# Autodesk Inventor assembly: PS MW RSP-2000-48
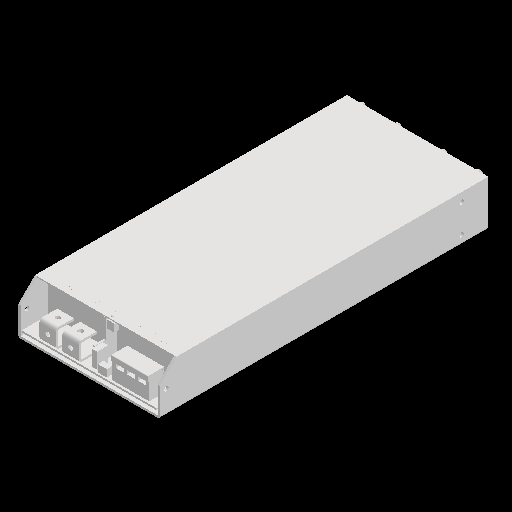
[picture p0: Inventor's stored thumbnail of the model, 512x512]
Saved by Autodesk Inventor 2025.2 (Build 292293000, 293)
## iProperties
Created: 2025-01-30
Part Number: PS MW RSP-2000-48
Description: STEP AP203
Document SubType Name: Assembly
Designer: valer
Sending System: SolidWorks 2012
Preprocessor: SwSTEP 2.0
Title: PS MW RSP-2000-48.STEP
Revision Number: ANY
## Documents named in this file (7)
- C:\Users\valer\Desktop\str1ker\cad\external\PowerSupply\MW RSP-2000-24.iam
- C:\Users\valer\Desktop\str1ker\cad\external\PowerSupply\Case PS RSP-2000-24.ipt
- C:\Users\valer\Desktop\str1ker\cad\external\PowerSupply\Terminal.ipt
- C:\Users\valer\Desktop\str1ker\cad\external\PowerSupply\Fan 40x40x28.ipt
- C:\Users\valer\Desktop\str1ker\cad\external\PowerSupply\Fan screw.ipt
- C:\Users\valer\Desktop\str1ker\cad\external\PowerSupply\Fan Guard 40õ40 K-G04D02-4HA JAMICON.ipt
- C:\Users\valer\Desktop\str1ker\cad\external\PowerSupply\PS Shield.ipt
## Components (16 placed, 16 different names)
1. Case PS RSP-2000-48_1 — Flush:1
2. Terminal_2
3. Terminal_3
4. Fan 40x40x28_4
5. Fan 40x40x28_5
6. Fan screw_6
7. Fan screw_7
8. Fan screw_8
9. Fan screw_9
10. Fan screw_10
11. Fan screw_11
12. Fan screw_12
13. Fan screw_13
14. Fan Guard 40õ40 K-G04D02-4HA JAMICON_14
15. Fan Guard 40õ40 K-G04D02-4HA JAMICON_15
16. PS Shield_16
## Relationships (1: Flush 1)
- Flush:1 (-63.5 mm): Case PS RSP-2000-48_1
